# Autodesk Inventor assembly: Telescope
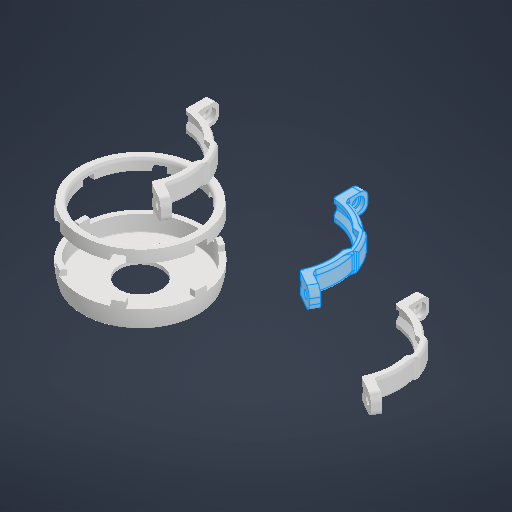
[picture p0: Inventor's stored thumbnail of the model, 512x512]
Saved by Autodesk Inventor 2026.2 (Build 302298010, 298A)
## iProperties
Created: 2026-03-08
Part Number: Telescope
Document SubType Name: Assembly
Designer: August
Author: August
## Documents named in this file (4)
- C:\Workspace\Telescope\Telescope.iam
- C:\Workspace\Telescope\Mirror_Housing_Bottom.ipt
- C:\Workspace\Telescope\Mirror_Housing_Top.ipt
- C:\Workspace\Telescope\Clamping_Ring.ipt
## Components (5 placed, 3 different names)
1. Mirror_Housing_Bottom:1 — Mate:1
2. Mirror_Housing_Top:1 — Mate:1, Mate:2
3. Clamping_Ring:1 — Mate:2
4. Clamping_Ring:2
5. Clamping_Ring:3
## Relationships (2: Mate 2)
- Mate:1: Mirror_Housing_Bottom:1 ↔ Mirror_Housing_Top:1
- Mate:2: Mirror_Housing_Top:1 ↔ Clamping_Ring:1
